# Autodesk Inventor assembly: Reactor Rod Holder Positions
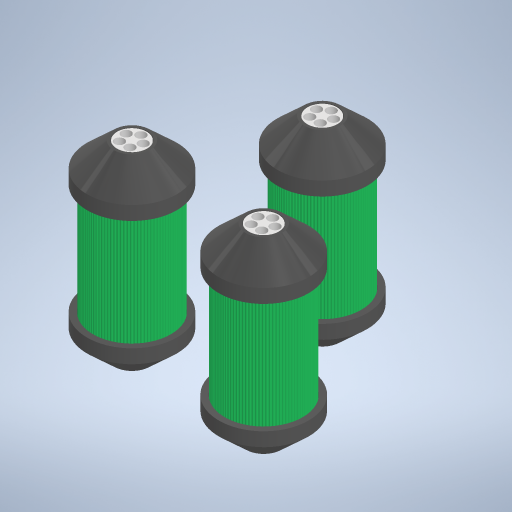
[picture p0: Inventor's stored thumbnail of the model, 512x512]
Saved by Autodesk Inventor 2024 (Build 280153020, 153B)
## iProperties
Created: 2023-08-02
Part Number: Reactor Rod Holder Positions
Document SubType Name: Assembly
Designer: torban
Author: torban
## Documents named in this file (2)
- D:\GIT\CIRC-2023-Night-Task-HW-SW\CAD\Reactor Module\Reactor Module\Print V1\Reactor Rod Holder Positions.iam
- D:\GIT\CIRC-2023-Night-Task-HW-SW\CAD\Reactor Module\Reactor Module\Final.iam
## Components (3 placed, 1 different names)
1. Final:1 [sub-assembly] — Flush:1, Flush:2, Mate:1, Mate:2
2. Final:2 [sub-assembly] — Flush:2, Mate:2, Mate:3
3. Final:3 [sub-assembly] — Flush:1, Mate:1, Mate:3
## Relationships (5: Mate 3, Flush 2)
- Flush:1: Final:1 ↔ Final:3
- Flush:2: Final:1 ↔ Final:2
- Mate:1 (100 mm): Final:1 ↔ Final:3
- Mate:2 (100 mm): Final:1 ↔ Final:2
- Mate:3 (100 mm): Final:2 ↔ Final:3
